# Autodesk Inventor assembly: gimbal_assembly
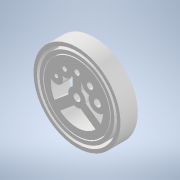
[picture p0: Inventor's stored thumbnail of the model, 180x180]
Saved by Autodesk Inventor 2021 (Build 250183000, 183)
## iProperties
Created: 2021-06-14
Part Number: gimbal_assembly
Document SubType Name: Assembly
Designer: Charlie
Author: Charlie
## Documents named in this file (4)
- C:\Users\Charlie\Downloads\gimbal_assembly.iam
- C:\Users\Charlie\Downloads\gimbal_medium_ring.ipt
- C:\Users\Charlie\Downloads\gimbal_inner_ring.ipt
- C:\Users\Charlie\Downloads\probe_gimbal_prototype.ipt
## Components (3 placed, 3 different names)
1. gimbal_medium_ring:1 — Mate:1, Mate:2
2. gimbal_inner_ring:1 — Mate:2
3. probe_gimbal_prototype:1 — Mate:1
## Relationships (2: Mate 2)
- Mate:1: gimbal_medium_ring:1 ↔ probe_gimbal_prototype:1
- Mate:2: gimbal_medium_ring:1 ↔ gimbal_inner_ring:1
